# Autodesk Inventor assembly: Tamale - v1p4b
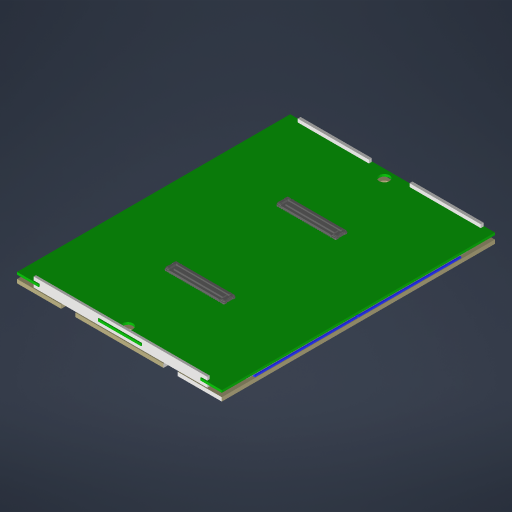
[picture p0: Inventor's stored thumbnail of the model, 512x512]
Saved by Autodesk Inventor 2024 (Build 280153000, 153)
## iProperties
Created: 2022-02-01
Part Number: Tamale - v1p4b
Document SubType Name: Assembly
Designer: Caleb
Author: Caleb
## Documents named in this file (8)
- C:\Users\cfangmeier3\Desktop\nebraska-silicon-lab\Hardware\ETL\modules\tamale v1.4\Tamale - v1p4b.iam
- C:\Users\cfangmeier3\Desktop\nebraska-silicon-lab\Hardware\ETL\modules\tamale v1.4\BBM.iam
- C:\Users\cfangmeier3\Desktop\nebraska-silicon-lab\Hardware\ETL\modules\tamale v1.4\Wirebond.ipt
- C:\Users\cfangmeier3\Desktop\nebraska-silicon-lab\Hardware\ETL\modules\tamale v1.4\Short Wirebond.ipt
- C:\Users\cfangmeier3\Desktop\nebraska-silicon-lab\Hardware\ETL\modules\tamale v1.4\Coverplate Film.ipt
- C:\Users\cfangmeier3\Desktop\nebraska-silicon-lab\Hardware\ETL\modules\tamale v1.4\Sensor Placement Film.ipt
- C:\Users\cfangmeier3\Desktop\nebraska-silicon-lab\Hardware\ETL\modules\tamale v1.4\Baseplate v1.4.ipt
- C:\Users\cfangmeier3\Desktop\nebraska-silicon-lab\Hardware\ETL\modules\tamale v1.4\Mock Module PCB - v1p4b.iam
## Components (150 placed, 7 different names)
1. BBM:1 [sub-assembly] — Mate:2, Angle:2, Flush:1, Flush:4, Mate:5, Flush:11
2. BBM:2 [sub-assembly] — Mate:3, Angle:1, Flush:2, Flush:4
3. BBM:3 [sub-assembly] — Mate:1, Angle:3, Flush:1, Flush:3, Mate:5, Mate:6, Flush:12
4. BBM:4 [sub-assembly] — Mate:4, Angle:4, Flush:2, Flush:3, Mate:6, Mate:10, Mate:11, Flush:9, Flush:10, Flush:14
5. Mock Module PCB - v1p4b:1 [sub-assembly] — Mate:1, Mate:2, Mate:3, Mate:4, Angle:1, Angle:2, Angle:3, Angle:4, Flush:11, Flush:15, Flush:16
6. Coverplate Film:1 — Mate:10, Flush:12, Flush:14, Mate:12
7. Sensor Placement Film:1 — Mate:11, Flush:9, Flush:10
8. Baseplate v1.4:1 — Mate:12, Flush:15, Flush:16
9. Wirebond:143
10. Wirebond:144
11. Wirebond:145
12. Wirebond:146
13. Wirebond:147
14. Wirebond:148
15. Wirebond:149
16. Wirebond:150
17. Wirebond:151
18. Wirebond:152
19. Wirebond:153
20. Wirebond:154
21. Wirebond:155
22. Wirebond:156
23. Wirebond:157
24. Wirebond:158
25. Wirebond:159
26. Wirebond:160
27. Wirebond:161
28. Wirebond:162
29. Wirebond:163
30. Wirebond:164
31. Wirebond:165
32. Wirebond:166
33. Wirebond:167
34. Wirebond:168
35. Wirebond:169
36. Wirebond:170
37. Wirebond:171
38. Wirebond:172
39. Wirebond:173
40. Wirebond:174
41. Wirebond:175
42. Wirebond:176
43. Wirebond:177
44. Wirebond:178
45. Wirebond:179
46. Wirebond:180
47. Wirebond:181
48. Wirebond:182
49. Wirebond:183
50. Wirebond:184
51. Wirebond:185
52. Wirebond:186
53. Wirebond:187
54. Wirebond:188
55. Wirebond:189
56. Wirebond:190
57. Wirebond:191
58. Wirebond:192
59. Wirebond:193
60. Wirebond:194
61. Wirebond:195
62. Wirebond:196
63. Wirebond:197
64. Wirebond:198
65. Wirebond:199
66. Wirebond:200
67. Wirebond:201
68. Wirebond:202
69. Wirebond:203
70. Wirebond:204
71. Wirebond:205
72. Wirebond:206
73. Wirebond:207
74. Wirebond:208
75. Wirebond:209
76. Wirebond:210
77. Wirebond:211
78. Wirebond:212
79. Wirebond:213
80. Short Wirebond:1
81. Short Wirebond:2
82. Short Wirebond:3
83. Short Wirebond:4
84. Short Wirebond:5
85. Short Wirebond:6
86. Short Wirebond:7
87. Short Wirebond:8
88. Short Wirebond:9
89. Short Wirebond:10
90. Short Wirebond:11
91. Short Wirebond:12
92. Short Wirebond:13
93. Short Wirebond:14
94. Short Wirebond:15
95. Short Wirebond:16
96. Short Wirebond:17
97. Short Wirebond:18
98. Short Wirebond:19
99. Short Wirebond:20
100. Short Wirebond:21
101. Short Wirebond:22
102. Short Wirebond:23
103. Short Wirebond:24
104. Short Wirebond:25
105. Short Wirebond:26
106. Short Wirebond:27
107. Short Wirebond:28
108. Short Wirebond:29
109. Short Wirebond:30
110. Short Wirebond:31
111. Short Wirebond:32
112. Short Wirebond:33
113. Short Wirebond:34
114. Short Wirebond:35
115. Short Wirebond:36
116. Short Wirebond:37
117. Short Wirebond:38
118. Short Wirebond:39
119. Short Wirebond:40
120. Short Wirebond:41
121. Short Wirebond:42
122. Short Wirebond:43
123. Short Wirebond:44
124. Short Wirebond:45
125. Short Wirebond:46
126. Short Wirebond:47
127. Short Wirebond:48
128. Short Wirebond:49
129. Short Wirebond:50
130. Short Wirebond:51
131. Short Wirebond:52
132. Short Wirebond:53
133. Short Wirebond:54
134. Short Wirebond:55
135. Short Wirebond:56
136. Short Wirebond:57
137. Short Wirebond:58
138. Short Wirebond:59
139. Short Wirebond:60
140. Short Wirebond:61
141. Short Wirebond:62
142. Short Wirebond:63
143. Short Wirebond:64
144. Short Wirebond:65
145. Short Wirebond:66
146. Short Wirebond:67
147. Short Wirebond:68
148. Short Wirebond:69
149. Short Wirebond:70
150. Short Wirebond:71
## Component patterns: (71 elements, first: Wirebond:143), (71 elements, first: Short Wirebond:1)
## Relationships (24: Flush 11, Mate 9, Angle 4)
- Mate:1 (0.08 mm): BBM:3 ↔ Mock Module PCB - v1p4b:1
- Mate:2 (0.08 mm): BBM:1 ↔ Mock Module PCB - v1p4b:1
- Mate:3 (0.08 mm): BBM:2 ↔ Mock Module PCB - v1p4b:1
- Mate:4 (0.08 mm): BBM:4 ↔ Mock Module PCB - v1p4b:1
- Angle:1 (0 deg): BBM:2 ↔ Mock Module PCB - v1p4b:1
- Angle:2 (0 deg): BBM:1 ↔ Mock Module PCB - v1p4b:1
- Angle:3 (0 deg): BBM:3 ↔ Mock Module PCB - v1p4b:1
- Angle:4 (0 deg): BBM:4 ↔ Mock Module PCB - v1p4b:1
- Flush:1: BBM:1 ↔ BBM:3
- Flush:2: BBM:2 ↔ BBM:4
- Flush:3: BBM:3 ↔ BBM:4
- Flush:4: BBM:1 ↔ BBM:2
- Mate:5 (0.2 mm): BBM:1 ↔ BBM:3
- Mate:6 (0.2 mm): BBM:3 ↔ BBM:4
- Mate:10: BBM:4 ↔ Coverplate Film:1
- Mate:11: BBM:4 ↔ Sensor Placement Film:1
- Flush:9: BBM:4 ↔ Sensor Placement Film:1
- Flush:10: BBM:4 ↔ Sensor Placement Film:1
- Flush:11 (0.25 mm): BBM:1 ↔ Mock Module PCB - v1p4b:1
- Flush:12 (0.5 mm): BBM:3 ↔ Coverplate Film:1
- Flush:14 (0.9 mm): BBM:4 ↔ Coverplate Film:1
- Mate:12: Coverplate Film:1 ↔ Baseplate v1.4:1
- Flush:15: Mock Module PCB - v1p4b:1 ↔ Baseplate v1.4:1
- Flush:16: Mock Module PCB - v1p4b:1 ↔ Baseplate v1.4:1
